# Autodesk Inventor assembly: Bottomplate2 assy1
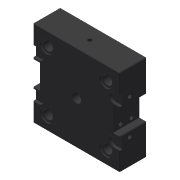
[picture p0: Inventor's stored thumbnail of the model, 180x180]
Saved by Autodesk Inventor 2022 Beta2 (Build 260130000, 130) ContinuousBuild 0
## iProperties
Shininess: 64.0
Length Units: 11272
Angle Units: 11279
Time Units: 11290
Mass Units: 11286
Length Display Precision: 3
Angle Display Precision: 2
Compacted: True
Part Number: Bottomplate2 assy1
Document SubType Name: Assembly
Created: 2003-04-07
Designer: demo
Density: 0.0
Volumn: 0.0
Area: 0.0
PropertySet Name: Model Information
Control State: 0
Master: False
Checked Out: False
Author: demo
## Documents named in this file (4)
- C:\Autodesk Inventor 2021 Intro Practice Files\Mold Assembly\Bottomplate2 assy1.iam
- C:\Autodesk Inventor 2021 Intro Practice Files\Mold Assembly\bottomplate2.ipt
- C:\Autodesk Inventor 2021 Intro Practice Files\Mold Assembly\cavity-bottom2.ipt
- C:\Autodesk Inventor 2021 Intro Practice Files\Mold Assembly\Bush bottomplate2.ipt
## Components (6 placed, 3 different names)
1. bottomplate2:1 — Mate:1, Flush:1, Mate:2
2. cavity-bottom2:1 — Mate:1, Flush:1
3. Bush bottomplate2:1 — Mate:2
4. Bush bottomplate2:2
5. Bush bottomplate2:3
6. Bush bottomplate2:4
## Component patterns: (4 elements, first: Bush bottomplate2:1)
## Relationships (3: Mate 2, Flush 1)
- Mate:1: bottomplate2:1 ↔ cavity-bottom2:1
- Flush:1: bottomplate2:1 ↔ cavity-bottom2:1
- Mate:2: bottomplate2:1 ↔ Bush bottomplate2:1
